# Autodesk Inventor assembly: Drive Body
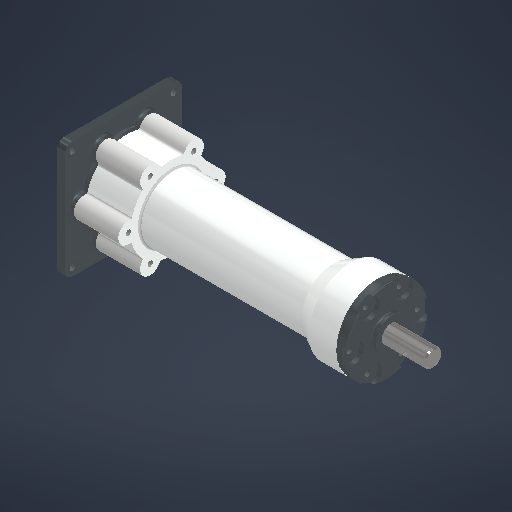
[picture p0: Inventor's stored thumbnail of the model, 512x512]
Saved by Autodesk Inventor 2026.1 (Build 301233020, 233B)
## iProperties
Created: 2025-10-14
Part Number: Drive Body
Document SubType Name: Assembly
Designer: Alexander
Author: Alexander
## Documents named in this file (9)
- C:\Users\Alexander\Documents\M&M Engineering Second year\Semester 2\Introductory Machine Design 254\Theory of Machines\Project\Part 2\Drive Body.iam
- C:\Users\Alexander\Documents\M&M Engineering Second year\Semester 2\Introductory Machine Design 254\Theory of Machines\Project\Part 2\Body.ipt
- C:\Users\Alexander\Documents\M&M Engineering Second year\Semester 2\Introductory Machine Design 254\Theory of Machines\Project\Part 2\Shaft.ipt
- C:\Users\Alexander\Documents\Inventor\Content Center Files\R2026\en-US\ISO 6194_1(2)\ISO 6194_1 - 25x47x7-Type 2.ipt
- C:\Users\Alexander\Documents\M&M Engineering Second year\Semester 2\Introductory Machine Design 254\Theory of Machines\Project\Part 2\Drive Body\Design Accelerator\Bearing2.iam
- C:\Users\Alexander\Documents\M&M Engineering Second year\Semester 2\Introductory Machine Design 254\Theory of Machines\Project\Part 2\END CAP.ipt
- C:\Users\Alexander\Documents\M&M Engineering Second year\Semester 2\Introductory Machine Design 254\Theory of Machines\Project\Part 2\Drive Body\Design Accelerator\Bearing3.iam
- C:\Users\Alexander\Documents\M&M Engineering Second year\Semester 2\Introductory Machine Design 254\Theory of Machines\Project\Part 2\BASE COVER.ipt
- C:\Users\Alexander\Documents\Inventor\Content Center Files\R2026\en-US\DIN 471(1)\DIN 471 - 25x1.2.ipt
## Components (9 placed, 7 different names)
1. Body:1 — Mate:2, Mate:23, Mate:24, Mate:27
2. Shaft:1 — Mate:2, Mate:10, Mate:18, Mate:19, Mate:22, Insert:1, Flush:1, Mate:25
3. ISO 6194/1 25x47x7-Type 2:1 — Mate:13, Flush:1
4. Bearing:1 [sub-assembly] — Mate:10, Mate:13, Mate:26
5. END CAP:1 — Mate:25, Mate:26, Mate:27
6. Bearing:2 [sub-assembly] — Mate:18, Mate:19, Mate:20, Mate:21
7. ISO 6194/1 25x47x7-Type 2:2 — Mate:20, Mate:21
8. BASE COVER:1 — Mate:22, Mate:23, Mate:24
9. DIN 471 25x1.2:1 — Insert:1
## Relationships (15: Mate 13, Insert 1, Flush 1)
- Mate:2: Body:1 ↔ Shaft:1
- Mate:10: Shaft:1 ↔ Bearing:1
- Mate:13: ISO 6194/1 25x47x7-Type 2:1 ↔ Bearing:1
- Mate:18 (3 mm): Shaft:1 ↔ Bearing:2
- Mate:19: Shaft:1 ↔ Bearing:2
- Mate:20 (2 mm): Bearing:2 ↔ ISO 6194/1 25x47x7-Type 2:2
- Mate:21: Bearing:2 ↔ ISO 6194/1 25x47x7-Type 2:2
- Mate:22: Shaft:1 ↔ BASE COVER:1
- Mate:23: Body:1 ↔ BASE COVER:1
- Mate:24: Body:1 ↔ BASE COVER:1
- Insert:1: Shaft:1 ↔ DIN 471 25x1.2:1
- Flush:1: Shaft:1 ↔ ISO 6194/1 25x47x7-Type 2:1
- Mate:25: Shaft:1 ↔ END CAP:1
- Mate:26: Bearing:1 ↔ END CAP:1
- Mate:27: Body:1 ↔ END CAP:1
